# Autodesk Inventor assembly: wing
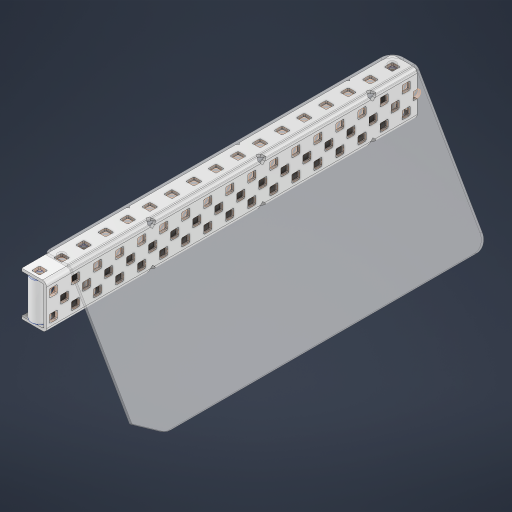
[picture p0: Inventor's stored thumbnail of the model, 512x512]
Saved by Autodesk Inventor 2024 (Build 280153000, 153)
## iProperties
Created: 2024-01-16
Part Number: wing
Document SubType Name: Assembly
Designer: avere
Author: avere
## Documents named in this file (4)
- C:\Users\avere\Documents\rbp_cad\zoomba_v0.3\chassis\drivebay\wing.iam
- C:\Users\avere\Documents\rbp_cad\VEX-CAD-Inventor-1.41\Structure\C Channel\Aluminum 1x2x1\Alu C 1x2x1x17.ipt
- C:\Users\avere\Documents\rbp_cad\hardware\.375 OD Aluminum Spacer 0.875.ipt
- C:\Users\avere\Documents\rbp_cad\zoomba_v0.3\chassis\drivebay\custom_parts\wing_wedge.ipt
## Components (5 placed, 3 different names)
1. Alu C 1x2x1x17:1 — Insert:1, Mate:1, Insert:3, Insert:4, Insert:5
2. .375 OD Aluminum Spacer 0.875:1 — Insert:1
3. wing_wedge:1 — Mate:1, Insert:4
4. .375 OD Aluminum Spacer 0.875:2 — Insert:3
5. .375 OD Aluminum Spacer 0.875:3 — Insert:5
## Relationships (5: Insert 4, Mate 1)
- Insert:1: Alu C 1x2x1x17:1 ↔ .375 OD Aluminum Spacer 0.875:1
- Mate:1: Alu C 1x2x1x17:1 ↔ wing_wedge:1
- Insert:3: Alu C 1x2x1x17:1 ↔ .375 OD Aluminum Spacer 0.875:2
- Insert:4: Alu C 1x2x1x17:1 ↔ wing_wedge:1
- Insert:5: Alu C 1x2x1x17:1 ↔ .375 OD Aluminum Spacer 0.875:3
